# Autodesk Inventor assembly: RatchetStrap
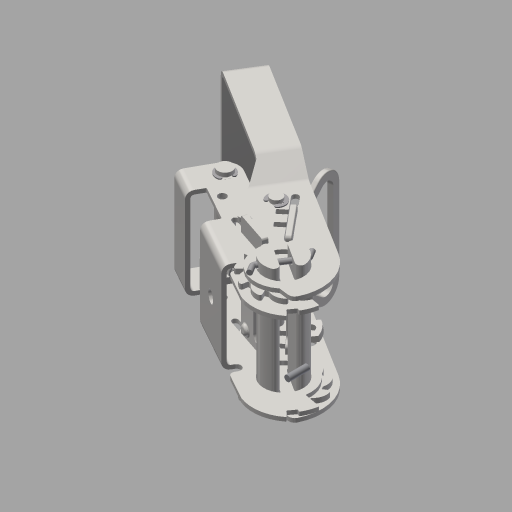
[picture p0: Inventor's stored thumbnail of the model, 512x512]
Saved by Autodesk Inventor 2023.2 (Build 272271000, 271)
## iProperties
Company: Summit Trailer Sales
Created: 2016-02-01
Part Number: RatchetStrap
Material: Generisch
Document SubType Name: Assembly
Designer: Raoul Messerli
Sending System: Autodesk Inventor 2016
Preprocessor: ST-DEVELOPER v16.1
Title: W:\Projects\Valley Protein\RatchetStrap.stp
Author: stuser
Revision Number: ANY
## Documents named in this file (14)
- E:\GitHub\Pflanzenwagen\20_Inventor\20_Einkaufteile\RatchetStrap\RatchetStrap\RatchetStrap.iam
- E:\GitHub\Pflanzenwagen\20_Inventor\20_Einkaufteile\RatchetStrap\rct.ipt
- E:\GitHub\Pflanzenwagen\20_Inventor\20_Einkaufteile\RatchetStrap\Part4^RatchetStrap.ipt
- E:\GitHub\Pflanzenwagen\20_Inventor\20_Einkaufteile\RatchetStrap\Latch1.ipt
- E:\GitHub\Pflanzenwagen\20_Inventor\20_Einkaufteile\RatchetStrap\Cross.ipt
- E:\GitHub\Pflanzenwagen\20_Inventor\20_Einkaufteile\RatchetStrap\Pin.ipt
- E:\GitHub\Pflanzenwagen\20_Inventor\20_Einkaufteile\RatchetStrap\Pin2.ipt
- E:\GitHub\Pflanzenwagen\20_Inventor\20_Einkaufteile\RatchetStrap\C_clip.ipt
- E:\GitHub\Pflanzenwagen\20_Inventor\20_Einkaufteile\RatchetStrap\MiddleBracket.ipt
- E:\GitHub\Pflanzenwagen\20_Inventor\20_Einkaufteile\RatchetStrap\DynamicSpring.ipt
- E:\GitHub\Pflanzenwagen\20_Inventor\20_Einkaufteile\RatchetStrap\Pin1.ipt
- E:\GitHub\Pflanzenwagen\20_Inventor\20_Einkaufteile\RatchetStrap\Gear.ipt
- E:\GitHub\Pflanzenwagen\20_Inventor\20_Einkaufteile\RatchetStrap\Latch2.ipt
- E:\GitHub\Pflanzenwagen\20_Inventor\20_Einkaufteile\RatchetStrap\Strap for Pflanzenwagen.ipt
## Components (18 placed, 18 different names)
1. rct_1
2. Part4^RatchetStrap_3
3. Latch1_4
4. Cross_5
5. Pin_6
6. Pin2_7
7. C_clip_8
8. Cross_9
9. Pin_11
10. MiddleBracket_12
11. DynamicSpring_13
12. C_clip_14
13. Pin1_15
14. Gear_16
15. C_clip_17
16. Gear_18
17. Latch2_19
18. Strap for Pflanzenwagen:1 — Passend:1, Passend:2, Fluchtend:1
## Relationships (3: Mate 2, Flush 1)
- Passend:1 [Mate]: Strap for Pflanzenwagen:1
- Passend:2 [Mate]: Strap for Pflanzenwagen:1
- Fluchtend:1 [Flush]: Strap for Pflanzenwagen:1
